# Autodesk Inventor assembly: 36mm Slim Tamiya
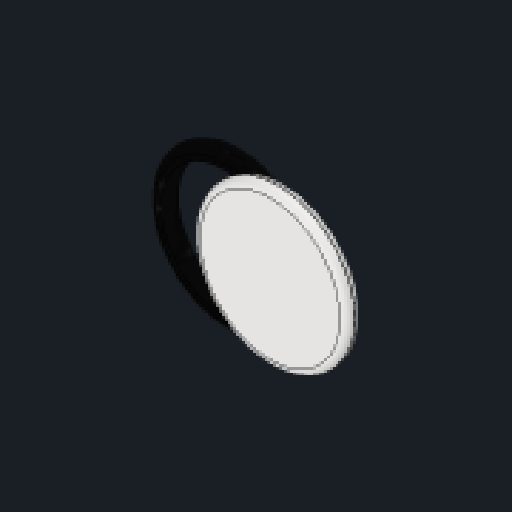
[picture p0: Inventor's stored thumbnail of the model, 512x512]
Saved by Autodesk Inventor 2023.2 (Build 272271030, 271C)
## iProperties
Created: 2024-02-20
Part Number: 36mm Slim Tamiya
Document SubType Name: Assembly
Designer: robpl
Author: robpl
## Documents named in this file (3)
- C:\Users\robpl\OneDrive\Documents\Arduino\Onslaught\CAD\tamiya-slim-tire-set-1.snapshot.2\36mm Slim Tamiya.iam
- C:\Users\robpl\OneDrive\Documents\Arduino\Onslaught\CAD\tamiya-slim-tire-set-1.snapshot.2\36mm tamiya-slim-tire-gomu.ipt
- C:\Users\robpl\OneDrive\Documents\Arduino\Onslaught\CAD\tamiya-slim-tire-set-1.snapshot.2\36mm tamiya-slim-tire-wheel.ipt
## Components (2 placed, 2 different names)
1. 36mm tamiya-slim-tire-gomu:1 — Mate:1, Mate:2
2. 36mm tamiya-slim-tire-wheel:1 — Mate:1, Mate:2
## Relationships (2: Mate 2)
- Mate:1: 36mm tamiya-slim-tire-gomu:1 ↔ 36mm tamiya-slim-tire-wheel:1
- Mate:2: 36mm tamiya-slim-tire-gomu:1 ↔ 36mm tamiya-slim-tire-wheel:1
